# Autodesk Inventor assembly: openmv4_h7
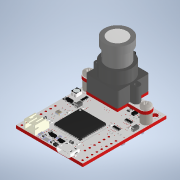
[picture p0: Inventor's stored thumbnail of the model, 180x180]
Saved by Autodesk Inventor 2020 (Build 240168000, 168)
## iProperties
Created: 2019-09-24
Part Number: openmv4_h7
Description: STEP AP214
Document SubType Name: Assembly
Designer: 4s
Sending System: SolidWorks 2016
Preprocessor: SwSTEP 2.0
Title: openmv4_h7.STEP
Revision Number: ANY
## Documents named in this file (7)
- C:\Users\4s\Documents\Inventor models\Asterisk\robot_v2\openmv\openmv4_h7.iam
- C:\Users\4s\Documents\Inventor models\Asterisk\robot_v2\openmv\openmv4_h7_base_® ã¬®«ç ­¨î.iam
- C:\Users\4s\Documents\Inventor models\Asterisk\robot_v2\openmv\openmv4_ov7725_® ã¬®«ç ­¨î.iam
- C:\Users\4s\Downloads\microsd card.ipt
- C:\Users\4s\Documents\Inventor models\Asterisk\robot_v2\openmv\LENS_Standard_® ã¬®«ç ­¨î.ipt
- C:\Users\4s\Downloads\LENS_Wide_® ã¬®«ç ­¨î.ipt
- C:\Users\4s\Downloads\Micro USB connector.ipt
## Components (6 placed, 6 different names)
1. openmv4_h7_base_® ã¬®«ç ­¨î_1 [sub-assembly] — Совмещение:3, Совмещение:4, Совмещение:5
2. openmv4_ov7725_® ã¬®«ç ­¨î_2 [sub-assembly] — Совмещение:1, Совмещение:2, Совмещение:3, Совмещение:4, Совмещение:5
3. microsd card_5
4. LENS_Standard_® ã¬®«ç ­¨î_6 — Совмещение:1, Совмещение:2
5. LENS_Wide_® ã¬®«ç ­¨î_7
6. Micro USB connector_8
## Relationships (5: Mate 5)
- Совмещение:1 [Mate]: openmv4_ov7725_® ã¬®«ç ­¨î_2 ↔ LENS_Standard_® ã¬®«ç ­¨î_6
- Совмещение:2 [Mate] (2 mm): openmv4_ov7725_® ã¬®«ç ­¨î_2 ↔ LENS_Standard_® ã¬®«ç ­¨î_6
- Совмещение:3 [Mate]: openmv4_h7_base_® ã¬®«ç ­¨î_1 ↔ openmv4_ov7725_® ã¬®«ç ­¨î_2
- Совмещение:4 [Mate]: openmv4_h7_base_® ã¬®«ç ­¨î_1 ↔ openmv4_ov7725_® ã¬®«ç ­¨î_2
- Совмещение:5 [Mate]: openmv4_h7_base_® ã¬®«ç ­¨î_1 ↔ openmv4_ov7725_® ã¬®«ç ­¨î_2
